# Autodesk Inventor assembly: 446 idler shaft
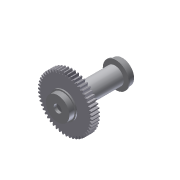
[picture p0: Inventor's stored thumbnail of the model, 180x180]
Saved by Autodesk Inventor 2013 (Build 170138000, 138)
## iProperties
Created: 2012-10-14
Part Number: 446 idler shaft
Document SubType Name: Assembly
Designer: Nemo
Author: Nemo
## Documents named in this file (5)
- H:\Nemo\Documents\Robotics\COTS Parts\Gearboxes\Shafts\446 idler shaft.iam
- H:\Nemo\Documents\Robotics\COTS Parts\Gearboxes\Shafts\AM Shifter Cluster Shaft.ipt
- H:\Nemo\Documents\Robotics\COTS Parts\Gearboxes\Bearings\Bearing 375 ID 1125 OD flanged.ipt
- H:\Nemo\Documents\Robotics\COTS Parts\Gearboxes\Gears\Gear 20dp 375hex 50T.ipt
- H:\Nemo\Documents\Robotics\COTS Parts\Gearboxes\Spacers\446 spacer for 375 hex.ipt
## Components (5 placed, 4 different names)
1. AM Shifter Cluster Shaft:1 — Insert:1, Mate:1, Mate:3, Angle:1, Mate:4
2. Bearing 375 ID 1125 OD flanged:1 — Insert:1, Mate:2
3. Bearing 375 ID 1125 OD flanged:2 — Mate:1, Mate:2
4. Gear 20dp 375hex 50T:1 — Mate:3, Angle:1
5. 446 spacer for 375 hex:1 — Mate:4
## Relationships (6: Mate 4, Insert 1, Angle 1)
- Insert:1: AM Shifter Cluster Shaft:1 ↔ Bearing 375 ID 1125 OD flanged:1
- Mate:1: AM Shifter Cluster Shaft:1 ↔ Bearing 375 ID 1125 OD flanged:2
- Mate:2 (-66.04 mm): Bearing 375 ID 1125 OD flanged:1 ↔ Bearing 375 ID 1125 OD flanged:2
- Mate:3: AM Shifter Cluster Shaft:1 ↔ Gear 20dp 375hex 50T:1
- Angle:1 (0 deg): AM Shifter Cluster Shaft:1 ↔ Gear 20dp 375hex 50T:1
- Mate:4: AM Shifter Cluster Shaft:1 ↔ 446 spacer for 375 hex:1
